# Autodesk Inventor assembly: rightSide
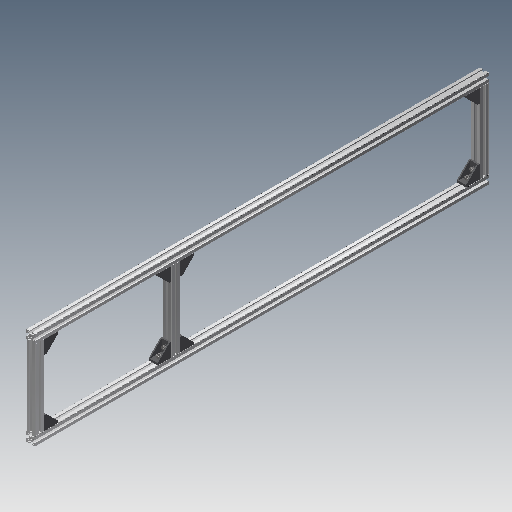
[picture p0: Inventor's stored thumbnail of the model, 512x512]
Saved by Autodesk Inventor 2017 (Build 210142000, 142)
## iProperties
Created: 2017-03-01
Part Number: rightSide
Document SubType Name: Assembly
Designer: sawaiz
Author: sawaiz
## Documents named in this file (5)
- C:\Users\sawaiz\oneDrive\projects\sPhenixTileTestStand\frame\rightSide.iam
- C:\Users\sawaiz\oneDrive\projects\sPhenixTileTestStand\frame\vertical.iam
- C:\Users\sawaiz\oneDrive\projects\sPhenixTileTestStand\frame\hfs5-2020Depth.ipt
- C:\Users\sawaiz\oneDrive\projects\sPhenixTileTestStand\hardware\angleBracket.iam
- C:\Users\sawaiz\oneDrive\projects\sPhenixTileTestStand\sPhenixTileTestStand.xlsx
## Components (13 placed, 3 different names)
1. vertical:1 [sub-assembly] — Flush:4, Flush:5, Flush:8, Mate:2, Mate:3, Flush:9, Flush:10, Flush:11, Flush:12, Mate:7
2. vertical:2 [sub-assembly] — Flush:3, Flush:5, Flush:6, Flush:7, Flush:8, Flush:13, Mate:6, Mate:8
3. vertical:3 [sub-assembly] — Flush:1, Mate:1, Flush:2, Flush:6, Flush:7, Flush:13, Mate:10
4. hfs5-2020Depth:1 — Symmetry:1, Symmetry:2, Symmetry:3, Mate:1, Flush:2, Mate:2, Flush:11, Flush:12, Flush:21, Mate:5, Mate:11
5. hfs5-2020Depth:2 — Symmetry:1, Symmetry:2, Symmetry:3, Flush:1, Flush:3, Flush:4, Mate:3, Flush:9, Flush:10, Mate:4, Mate:9
6. angleBracket:1 [sub-assembly] — Flush:14, Flush:15, Flush:28, Flush:29
7. angleBracket:2 [sub-assembly] — Flush:14, Flush:26, Flush:29, Mate:10, Mate:11
8. angleBracket:3 [sub-assembly] — Flush:16, Flush:17, Flush:26, Flush:27
9. angleBracket:4 [sub-assembly] — Flush:15, Flush:16, Flush:27, Flush:28, Mate:8, Mate:9
10. angleBracket:5 [sub-assembly] — Flush:18, Flush:19, Flush:23, Flush:24, Mate:4
11. angleBracket:6 [sub-assembly] — Flush:17, Flush:18, Flush:24, Flush:25, Mate:5, Mate:6
12. angleBracket:7 [sub-assembly] — Flush:20, Flush:21, Flush:22, Flush:25, Mate:7
13. angleBracket:8 [sub-assembly] — Flush:19, Flush:20, Flush:22, Flush:23
## Relationships (43: Flush 29, Mate 11, Symmetry 3)
- Symmetry:1: hfs5-2020Depth:1 ↔ hfs5-2020Depth:2
- Symmetry:2: hfs5-2020Depth:1 ↔ hfs5-2020Depth:2
- Symmetry:3: hfs5-2020Depth:1 ↔ hfs5-2020Depth:2
- Flush:1: vertical:3 ↔ hfs5-2020Depth:2
- Mate:1: vertical:3 ↔ hfs5-2020Depth:1
- Flush:2: vertical:3 ↔ hfs5-2020Depth:1
- Flush:3: vertical:2 ↔ hfs5-2020Depth:2
- Flush:4: vertical:1 ↔ hfs5-2020Depth:2
- Flush:5: vertical:1 ↔ vertical:2
- Flush:6: vertical:2 ↔ vertical:3
- Flush:7: vertical:2 ↔ vertical:3
- Flush:8: vertical:1 ↔ vertical:2
- Mate:2: vertical:1 ↔ hfs5-2020Depth:1
- Mate:3: vertical:1 ↔ hfs5-2020Depth:2
- Flush:9: vertical:1 ↔ hfs5-2020Depth:2
- Flush:10: vertical:1 ↔ hfs5-2020Depth:2
- Flush:11: vertical:1 ↔ hfs5-2020Depth:1
- Flush:12: vertical:1 ↔ hfs5-2020Depth:1
- Flush:13 (300 mm): vertical:2 ↔ vertical:3
- Flush:14: angleBracket:1 ↔ angleBracket:2
- Flush:15: angleBracket:1 ↔ angleBracket:4
- Flush:16: angleBracket:3 ↔ angleBracket:4
- Flush:17: angleBracket:3 ↔ angleBracket:6
- Flush:18: angleBracket:5 ↔ angleBracket:6
- Flush:19: angleBracket:5 ↔ angleBracket:8
- Flush:20: angleBracket:7 ↔ angleBracket:8
- Flush:21: hfs5-2020Depth:1 ↔ angleBracket:7
- Flush:22: angleBracket:7 ↔ angleBracket:8
- Flush:23: angleBracket:5 ↔ angleBracket:8
- Flush:24: angleBracket:5 ↔ angleBracket:6
- Flush:25: angleBracket:6 ↔ angleBracket:7
- Flush:26: angleBracket:2 ↔ angleBracket:3
- Flush:27: angleBracket:3 ↔ angleBracket:4
- Flush:28: angleBracket:1 ↔ angleBracket:4
- Flush:29: angleBracket:1 ↔ angleBracket:2
- Mate:4: hfs5-2020Depth:2 ↔ angleBracket:5
- Mate:5: hfs5-2020Depth:1 ↔ angleBracket:6
- Mate:6: vertical:2 ↔ angleBracket:6
- Mate:7: vertical:1 ↔ angleBracket:7
- Mate:8: vertical:2 ↔ angleBracket:4
- Mate:9: hfs5-2020Depth:2 ↔ angleBracket:4
- Mate:10: vertical:3 ↔ angleBracket:2
- Mate:11: hfs5-2020Depth:1 ↔ angleBracket:2
## Named parameters: plateWidth = 300 mm, plateDepth = 1000 mm, supportPlateThickness = 6.35 mm, supportPlateWidth = 50 mm, supportPlateFillet = 10 mm, separation = 35 mm, numPanels = 5, centerVerticalRatio = 0.3
